# Autodesk Inventor assembly: MontagemREV2 - Copia
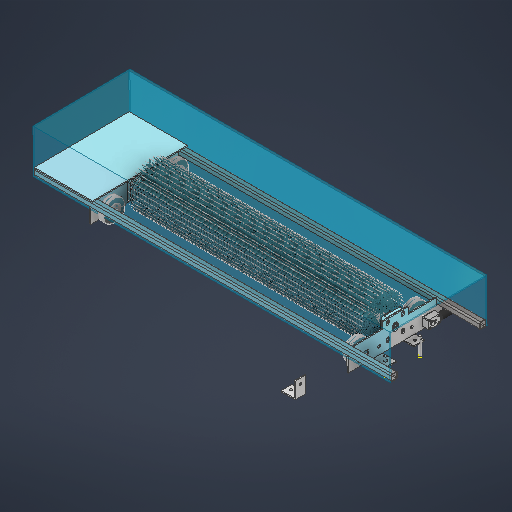
[picture p0: Inventor's stored thumbnail of the model, 512x512]
Saved by Autodesk Inventor 2026.1 (Build 301233020, 233B)
## iProperties
Created: 2025-11-04
Part Number: MontagemREV2 - Copia
Document SubType Name: Assembly
Designer: Rubens
Author: Rubens
## Documents named in this file (18)
- C:\Users\062210040\Downloads\TCC 1204\TCC 1204\TCC 1004\TCC 3103\TCC 3003\TCC 2903\TCC1803\TCC 1703\Projeto TCC\Projeto Limpador\MontagemREVXX.iam
- C:\Users\062210040\Downloads\TCC 1204\TCC 1204\TCC 1004\TCC 3103\TCC 3003\TCC 2903\TCC1803\TCC 1703\Projeto TCC\Projeto Limpador\Teste Suporte.ipt
- C:\Users\062210040\Downloads\TCC 1204\TCC 1204\TCC 1004\TCC 3103\TCC 3003\TCC 2903\TCC1803\TCC 1703\Projeto TCC\Projeto Limpador\TCC\Suporte Painel1.ipt
- C:\Users\062210040\Downloads\TCC 1204\TCC 1204\TCC 1004\TCC 3103\TCC 3003\TCC 2903\TCC1803\TCC 1703\Projeto TCC\Projeto Limpador\Teste Limpador.ipt
- C:\Users\062210040\Downloads\TCC 1204\TCC 1204\TCC 1004\TCC 3103\TCC 3003\TCC 2903\TCC1803\TCC 1703\Projeto TCC\Projeto Limpador\Suporte _ Motores.ipt
- C:\Users\062210040\Downloads\TCC 1204\TCC 1204\TCC 1004\TCC 3103\TCC 3003\TCC 2903\TCC1803\TCC 1703\Projeto TCC\Projeto Limpador\Proteção.ipt
- C:\Users\062210040\Downloads\TCC 1204\TCC 1204\TCC 1004\TCC 3103\TCC 3003\TCC 2903\TCC1803\TCC 1703\Projeto TCC\Projeto Limpador\Perfil 30X30 LIMPA.ipt
- C:\Users\062210040\Downloads\TCC 1204\TCC 1204\TCC 1004\TCC 3103\TCC 3003\TCC 2903\TCC1803\TCC 1703\Projeto TCC\Projeto Limpador\TCC\22874-100-g-a.ipt
- C:\Users\062210040\Downloads\TCC 1204\TCC 1204\TCC 1004\TCC 3103\TCC 3003\TCC 2903\TCC1803\TCC 1703\Projeto TCC\Projeto Limpador\TCC\Suporte painel 2.ipt
- C:\Users\062210040\Downloads\TCC 1204\TCC 1204\TCC 1004\TCC 3103\TCC 3003\TCC 2903\TCC1803\TCC 1703\Projeto TCC\Projeto Limpador\Orbit500-V2.0-64X-Motor555-Step\Orbit500-V2.0-64X-Motor555-Step\Orbit500-V2.0-64X-Motor555-Step.ipt
- C:\Users\062210040\Downloads\TCC 1204\TCC 1204\TCC 1004\TCC 3103\TCC 3003\TCC 2903\TCC1803\TCC 1703\Projeto TCC\Projeto Limpador\Worm_Gear_Motor_12V.ipt
- C:\Users\062210040\Downloads\painel-400-x-300-x-200-1.snapshot.1 (1)\Painel\00.PAINEL ELÉTRICO\00.PAINEL ELÉTRICO\00.PAINEL ELÉTRICO_TOP.iam
- C:\Users\062210040\Downloads\TCC 1204\TCC 1204\TCC 1004\TCC 3103\TCC 3003\TCC 2903\TCC1803\TCC 1703\Projeto TCC\Main_Solar_Structure\snr_sesf205-16coe_0.ipt
- C:\Users\062210040\Downloads\TCC 1204\TCC 1204\Eixo.ipt
- C:\Users\062210040\Documents\Inventor\Content Center Files\R2026\en-US\BS EN ISO 4762\BS EN ISO 4762 - M12 x 40(1).ipt
- C:\Users\062210040\Downloads\TCC 1204\TCC 1204\Componentes\Componentes\jlcmc-shaft-couplings-jaw-coupling-spider-type-elastomer-coupling-1.snapshot.1\CXHG-C-D25-d5-e8\CXHG-C-D25-d5-e8\CXHG-C-D25-d5-e8.iam
- C:\Users\062210040\Downloads\Escova.ipt
- C:\Users\062210040\Downloads\Suporte _ Motoresrev3\Suporte _ Motoresrev3\Suporte _ Motoresrev3.ipt
## Components (40 placed, 17 different names)
1. Teste Limpador:2
2. Perfil 30X30 LIMPA:3 — Mate:118, Mate:121, Flush:18, Flush:19, Flush:20, Mate:146, Flush:25, Flush:26, Flush:27, Flush:30, Flush:35, Flush:40
3. Perfil 30X30 LIMPA:4 — Mate:119, Mate:120, Mate:152, Flush:23, Flush:24, Flush:28, Mate:157, Flush:30, Flush:35, Mate:235, Mate:236
4. Suporte _ Motores:4 — Mate:118, Mate:119, Mate:120, Mate:121, Flush:18, Mate:123, Mate:124, Mate:125, Angle:1, Angle:2, Mate:188, Mate:215, Mate:216, Mate:217, Mate:219, Flush:32, Mate:226, Mate:227, Mate:230, Flush:33, Mate:233
5. Teste Suporte:13 — Mate:199, Mate:200, Mate:209, Flush:39
6. Teste Suporte:14 — Mate:123, Mate:125, Angle:2, Mate:194, Mate:195, Mate:208, Mate:232, Flush:36
7. Teste Suporte:15 — Mate:124, Angle:1, Mate:188, Mate:196, Mate:197, Mate:204, Mate:207, Mate:232, Flush:37
8. Suporte Painel1:4 — Flush:19, Flush:20, Mate:146, Mate:172, Flush:29
9. Proteção:2 — Mate:152, Flush:23, Flush:24, Flush:25, Flush:26, Mate:158, Mate:173
10. Suporte painel 2:1 — Flush:27, Flush:28, Mate:157, Mate:158
11. 00.PAINEL ELÉTRICO_TOP:1 [sub-assembly] — Mate:172, Mate:173, Flush:29
12. Orbit500-V2.0-64X-Motor555-Step:2 — Mate:233
13. Eixo:1 — Mate:202
14. Eixo:2 — Mate:205, Flush:37
15. Eixo:3 — Mate:230, Flush:33
16. Eixo:4 — Mate:206, Flush:36
17. 22874-100-g-a:15 — Mate:194, Mate:195, Mate:206
18. 22874-100-g-a:16 — Mate:196, Mate:197, Mate:204, Mate:205
19. 22874-100-g-a:17 — Mate:202
20. 22874-100-g-a:18 — Mate:199, Mate:200, Mate:203
21. Eixo:5 — Mate:203, Flush:39
22. BS EN ISO 4762 - Metric M12 x 40:1 — Mate:207
23. BS EN ISO 4762 - Metric M12 x 40:2 — Mate:208
24. BS EN ISO 4762 - Metric M12 x 40:3
25. BS EN ISO 4762 - Metric M12 x 40:4 — Mate:209
26. Worm_Gear_Motor_12V:5 — Mate:225
27. Worm_Gear_Motor_12V:6 — Mate:224
28. 22874-100-g-a:19 — Mate:220, Mate:222, Mate:223
29. 22874-100-g-a:20 — Mate:221
30. snr_sesf205-16coe_0:7 — Mate:215, Mate:216, Mate:217
31. snr_sesf205-16coe_0:8 — Mate:237, Mate:238, Mate:239
32. CXHG-C-D25-d5-e8:1 [sub-assembly] — Mate:220, Mate:222, Mate:223, Mate:225, Mate:240
33. CXHG-C-D25-d5-e8:2 [sub-assembly] — Mate:219, Flush:32, Mate:221, Mate:224
34. 22874-100-g-a:21
35. 22874-100-g-a:22 — Mate:226, Mate:227
36. Escova:1 — Mate:239, Flush:41
37. Suporte _ Motoresrev3:1 — Mate:235, Mate:236, Flush:40, Mate:237, Mate:238, Flush:41, Mate:240, Mate:241, Mate:242, Mate:243, Mate:244
38. Teste Suporte:16 — Mate:241, Mate:242
39. Teste Suporte:17
40. Teste Suporte:18 — Mate:243, Mate:244
## Relationships (74: Mate 53, Flush 19, Angle 2)
- Mate:118: Perfil 30X30 LIMPA:3 ↔ Suporte _ Motores:4
- Mate:119: Perfil 30X30 LIMPA:4 ↔ Suporte _ Motores:4
- Mate:120: Perfil 30X30 LIMPA:4 ↔ Suporte _ Motores:4
- Mate:121: Perfil 30X30 LIMPA:3 ↔ Suporte _ Motores:4
- Flush:18 (255 mm): Perfil 30X30 LIMPA:3 ↔ Suporte _ Motores:4
- Mate:123: Suporte _ Motores:4 ↔ Teste Suporte:14
- Mate:124: Suporte _ Motores:4 ↔ Teste Suporte:15
- Mate:125: Suporte _ Motores:4 ↔ Teste Suporte:14
- Flush:19: Perfil 30X30 LIMPA:3 ↔ Suporte Painel1:4
- Flush:20: Perfil 30X30 LIMPA:3 ↔ Suporte Painel1:4
- Mate:146: Perfil 30X30 LIMPA:3 ↔ Suporte Painel1:4
- Mate:152: Perfil 30X30 LIMPA:4 ↔ Proteção:2
- Flush:23: Perfil 30X30 LIMPA:4 ↔ Proteção:2
- Flush:24: Perfil 30X30 LIMPA:4 ↔ Proteção:2
- Flush:25: Perfil 30X30 LIMPA:3 ↔ Proteção:2
- Flush:26: Perfil 30X30 LIMPA:3 ↔ Proteção:2
- Flush:27: Perfil 30X30 LIMPA:3 ↔ Suporte painel 2:1
- Flush:28: Perfil 30X30 LIMPA:4 ↔ Suporte painel 2:1
- Mate:157: Perfil 30X30 LIMPA:4 ↔ Suporte painel 2:1
- Mate:158: Proteção:2 ↔ Suporte painel 2:1
- Angle:1 (0 deg): Suporte _ Motores:4 ↔ Teste Suporte:15
- Angle:2 (0 deg): Suporte _ Motores:4 ↔ Teste Suporte:14
- Mate:172: Suporte Painel1:4 ↔ 00.PAINEL ELÉTRICO_TOP:1
- Mate:173 (20 mm): Proteção:2 ↔ 00.PAINEL ELÉTRICO_TOP:1
- Flush:29: Suporte Painel1:4 ↔ 00.PAINEL ELÉTRICO_TOP:1
- Mate:188: Suporte _ Motores:4 ↔ Teste Suporte:15
- Mate:194: Teste Suporte:14 ↔ 22874-100-g-a:15
- Mate:195: Teste Suporte:14 ↔ 22874-100-g-a:15
- Mate:196: Teste Suporte:15 ↔ 22874-100-g-a:16
- Mate:197: Teste Suporte:15 ↔ 22874-100-g-a:16
- Mate:199: Teste Suporte:13 ↔ 22874-100-g-a:18
- Mate:200: Teste Suporte:13 ↔ 22874-100-g-a:18
- Mate:202: Eixo:1 ↔ 22874-100-g-a:17
- Mate:203: 22874-100-g-a:18 ↔ Eixo:5
- Mate:204: Teste Suporte:15 ↔ 22874-100-g-a:16
- Mate:205: Eixo:2 ↔ 22874-100-g-a:16
- Mate:206: Eixo:4 ↔ 22874-100-g-a:15
- Mate:207: Teste Suporte:15 ↔ BS EN ISO 4762 - Metric M12 x 40:1
- Mate:208: Teste Suporte:14 ↔ BS EN ISO 4762 - Metric M12 x 40:2
- Mate:209: Teste Suporte:13 ↔ BS EN ISO 4762 - Metric M12 x 40:4
- Flush:30: Perfil 30X30 LIMPA:3 ↔ Perfil 30X30 LIMPA:4
- Mate:215: Suporte _ Motores:4 ↔ snr_sesf205-16coe_0:7
- Mate:216: Suporte _ Motores:4 ↔ snr_sesf205-16coe_0:7
- Mate:217: Suporte _ Motores:4 ↔ snr_sesf205-16coe_0:7
- Mate:219: Suporte _ Motores:4 ↔ CXHG-C-D25-d5-e8:2
- Flush:32: Suporte _ Motores:4 ↔ CXHG-C-D25-d5-e8:2
- Mate:220: 22874-100-g-a:19 ↔ CXHG-C-D25-d5-e8:1
- Mate:221: 22874-100-g-a:20 ↔ CXHG-C-D25-d5-e8:2
- Mate:222: 22874-100-g-a:19 ↔ CXHG-C-D25-d5-e8:1
- Mate:223: 22874-100-g-a:19 ↔ CXHG-C-D25-d5-e8:1
- Mate:224: Worm_Gear_Motor_12V:6 ↔ CXHG-C-D25-d5-e8:2
- Mate:225: Worm_Gear_Motor_12V:5 ↔ CXHG-C-D25-d5-e8:1
- Mate:226: Suporte _ Motores:4 ↔ 22874-100-g-a:22
- Mate:227: Suporte _ Motores:4 ↔ 22874-100-g-a:22
- Mate:230: Suporte _ Motores:4 ↔ Eixo:3
- Flush:33 (20 mm): Suporte _ Motores:4 ↔ Eixo:3
- Mate:232: Teste Suporte:14 ↔ Teste Suporte:15
- Flush:35: Perfil 30X30 LIMPA:3 ↔ Perfil 30X30 LIMPA:4
- Flush:36 (-20 mm): Teste Suporte:14 ↔ Eixo:4
- Flush:37 (-20 mm): Teste Suporte:15 ↔ Eixo:2
- Flush:39 (-20 mm): Teste Suporte:13 ↔ Eixo:5
- Mate:233: Suporte _ Motores:4 ↔ Orbit500-V2.0-64X-Motor555-Step:2
- Mate:235: Perfil 30X30 LIMPA:4 ↔ Suporte _ Motoresrev3:1
- Mate:236: Perfil 30X30 LIMPA:4 ↔ Suporte _ Motoresrev3:1
- Flush:40 (200 mm): Perfil 30X30 LIMPA:3 ↔ Suporte _ Motoresrev3:1
- Mate:237: snr_sesf205-16coe_0:8 ↔ Suporte _ Motoresrev3:1
- Mate:238: snr_sesf205-16coe_0:8 ↔ Suporte _ Motoresrev3:1
- Mate:239: snr_sesf205-16coe_0:8 ↔ Escova:1
- Flush:41 (50 mm): Escova:1 ↔ Suporte _ Motoresrev3:1
- Mate:240: CXHG-C-D25-d5-e8:1 ↔ Suporte _ Motoresrev3:1
- Mate:241: Suporte _ Motoresrev3:1 ↔ Teste Suporte:16
- Mate:242 (20 mm): Suporte _ Motoresrev3:1 ↔ Teste Suporte:16
- Mate:243: Suporte _ Motoresrev3:1 ↔ Teste Suporte:18
- Mate:244 (20 mm): Suporte _ Motoresrev3:1 ↔ Teste Suporte:18
